# Autodesk Inventor assembly: FAN
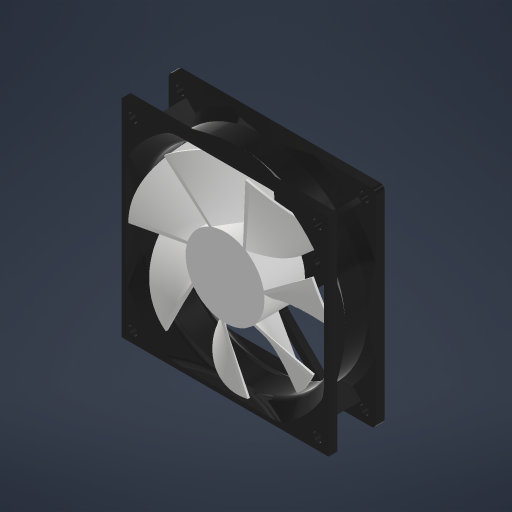
[picture p0: Inventor's stored thumbnail of the model, 512x512]
Saved by Autodesk Inventor 2024 (Build 280153000, 153)
## iProperties
Created: 2023-07-11
Part Number: FAN
Document SubType Name: Assembly
Designer: 6gioc
Author: 6gioc
## Documents named in this file (3)
- C:\Users\6gioc\OneDrive\AAST\PART\FAN.iam
- C:\Users\6gioc\OneDrive\AAST\PART\fancase.ipt
- C:\Users\6gioc\OneDrive\AAST\PART\FAN blade.ipt
## Components (2 placed, 2 different names)
1. fancase:1 — 회전:1
2. FAN blade:1 — 회전:1
## Relationships (1: RevoluteJoint 1)
- 회전:1 [RevoluteJoint]: fancase:1 ↔ FAN blade:1
